# Autodesk Inventor assembly: Lid Assembly
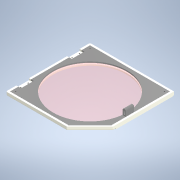
[picture p0: Inventor's stored thumbnail of the model, 180x180]
Saved by Autodesk Inventor 2022 (Build 260153000, 153)
## iProperties
Created: 2023-02-27
Part Number: Lid Assembly
Document SubType Name: Assembly
Designer: zarek
Author: zarek
## Documents named in this file (4)
- C:\Users\zarek\OneDrive\Desktop\Random New Stuff\SPB\Lid Parts\Lid Assembly.iam
- C:\Users\zarek\OneDrive\Desktop\Random New Stuff\SPB\Lid.ipt
- C:\Users\zarek\OneDrive\Desktop\Random New Stuff\SPB\Lid_Clear_Holder.ipt
- C:\Users\zarek\OneDrive\Desktop\Random New Stuff\SPB\Lid_Clear_Model.ipt
## Components (3 placed, 3 different names)
1. Lid:1 — Mate:1, Mate:2, Mate:3
2. Lid_Clear_Holder:1 — Mate:1, Mate:2, Mate:3
3. Lid_Clear_Model:1
## Relationships (3: Mate 3)
- Mate:1: Lid:1 ↔ Lid_Clear_Holder:1
- Mate:2: Lid:1 ↔ Lid_Clear_Holder:1
- Mate:3: Lid:1 ↔ Lid_Clear_Holder:1
